# Autodesk Inventor assembly: Сборка1
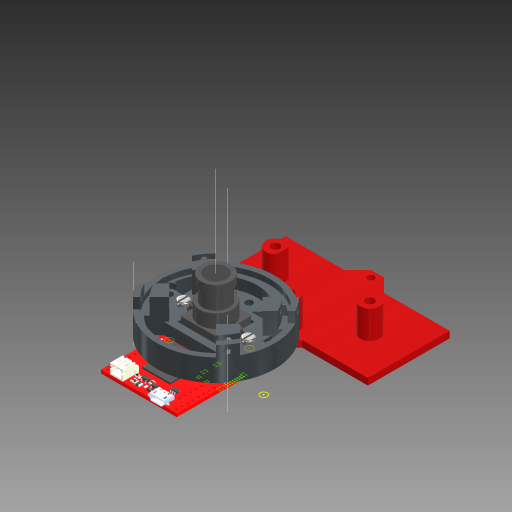
[picture p0: Inventor's stored thumbnail of the model, 512x512]
Saved by Autodesk Inventor 2023 (Build 270158000, 158)
## iProperties
Created: 2025-04-22
Part Number: Сборка1
Document SubType Name: Assembly
Designer: Ivan
Author: Ivan
## Documents named in this file (3)
- C:\!projects\dash_localDirectory\DASH_\Dash-V1\bashnia\Сборка1.iam
- C:\!projects\dash_localDirectory\DASH_\Dash-V1\step\akb_m\akb_mount1550V2B.ipt
- C:\!projects\dash_localDirectory\DASH_\Dash-V1\kamera_centre.iam
## Components (3 placed, 2 different names)
1. akb_mount1550V2B:1 — Совмещение:1, Совмещение:2, Заподлицо:1, Вставка:1, Вставка:2, Совмещение:3, Совмещение:6, Угол:1, Совмещение:7, Совмещение:8
2. kamera_centre:1 [sub-assembly] — Вставка:1, Вставка:2, Совмещение:3, Совмещение:4
3. kamera_centre:2 [sub-assembly] — Совмещение:5, Совмещение:6, Угол:1, Совмещение:7, Совмещение:8
## Relationships (12: Mate 8, Insert 2, Flush 1, Angle 1)
- Совмещение:1 [Mate]: akb_mount1550V2B:1
- Совмещение:2 [Mate]: akb_mount1550V2B:1
- Заподлицо:1 [Flush]: akb_mount1550V2B:1
- Вставка:1 [Insert]: akb_mount1550V2B:1 ↔ kamera_centre:1
- Вставка:2 [Insert]: akb_mount1550V2B:1 ↔ kamera_centre:1
- Совмещение:3 [Mate]: akb_mount1550V2B:1 ↔ kamera_centre:1
- Совмещение:4 [Mate]: kamera_centre:1
- Совмещение:5 [Mate]: kamera_centre:2
- Совмещение:6 [Mate]: akb_mount1550V2B:1 ↔ kamera_centre:2
- Угол:1 [Angle] (180 deg): akb_mount1550V2B:1 ↔ kamera_centre:2
- Совмещение:7 [Mate]: akb_mount1550V2B:1 ↔ kamera_centre:2
- Совмещение:8 [Mate]: akb_mount1550V2B:1 ↔ kamera_centre:2
